# Autodesk Inventor assembly: MagneticEncoder
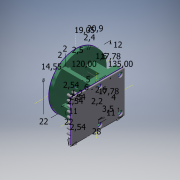
[picture p0: Inventor's stored thumbnail of the model, 180x180]
Saved by Autodesk Inventor 2019.1 (Build 231200000, 200)
## iProperties
Created: 2018-11-04
Part Number: MagneticEncoder
Material: Generisch
Document SubType Name: Assembly
Designer: JochenAlt
Author: JochenAlt
## Documents named in this file (5)
- D:\Projects\Ondine\CAD\Encoder\MagneticEncoder.iam
- D:\Projects\Ondine\CAD\Encoder\MagnetHolder.ipt
- D:\Projects\Ondine\CAD\Encoder\Magnet.ipt
- D:\Projects\Ondine\CAD\Encoder\AS5047D.ipt
- D:\Projects\Ondine\CAD\Encoder\AS5047DEnclosure.ipt
## Components (4 placed, 4 different names)
1. MagnetHolder:1 — Passend:6, Passend:7
2. Magnet:1 — Passend:6, Passend:7
3. AS5047D:1 — Passend:15, Passend:16
4. AS5047DEnclosure:1 — Passend:15, Passend:16
## Relationships (4: Mate 4)
- Passend:6 [Mate]: MagnetHolder:1 ↔ Magnet:1
- Passend:7 [Mate]: MagnetHolder:1 ↔ Magnet:1
- Passend:15 [Mate]: AS5047D:1 ↔ AS5047DEnclosure:1
- Passend:16 [Mate]: AS5047D:1 ↔ AS5047DEnclosure:1
